# Autodesk Inventor assembly: Raspberry Pi 3 Case
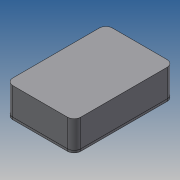
[picture p0: Inventor's stored thumbnail of the model, 180x180]
Saved by Autodesk Inventor 2016 SP2 (Build 200236200, 236)
## iProperties
Created: 2016-10-24
Part Number: Raspberry Pi 3 Case
Material: Generisch
Document SubType Name: Assembly
Designer: BU
Mass: 34.5987 g
Surface Area: 363.416 cm^2
Volume: 34.5987 cm^3
Density: 1 g/cm^3
Author: BU
Revision Number: -
## Documents named in this file (3)
- C:\Users\andreas.bauer\Desktop\Raspberry Pi 3 Case.iam
- C:\Users\andreas.bauer\Desktop\00002832.ipt
- C:\Users\andreas.bauer\Desktop\Bauteil8.ipt
## Components (2 placed, 2 different names)
1. 00002832:1 — Passend:1, Fluchtend:2, Passend:2
2. Bauteil8:1 — Passend:1, Fluchtend:2, Passend:2
## Relationships (3: Mate 2, Flush 1)
- Passend:1 [Mate]: 00002832:1 ↔ Bauteil8:1
- Fluchtend:2 [Flush]: 00002832:1 ↔ Bauteil8:1
- Passend:2 [Mate]: 00002832:1 ↔ Bauteil8:1
